# Autodesk Inventor assembly: 1001_Bias_Coil_Holder_MPSv2_v2
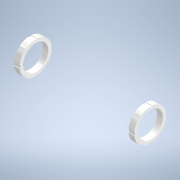
[picture p0: Inventor's stored thumbnail of the model, 180x180]
Saved by Autodesk Inventor 2021 (Build 250183000, 183)
## iProperties
Created: 2020-11-17
Part Number: 1001_Bias_Coil_Holder_MPSv2_v2
Document SubType Name: Assembly
Designer: Admin
Author: Admin
## Documents named in this file (3)
- C:\Users\Barksdale\Dropbox (MIT)\MPI Group Folder\MPS\Inventor_Parts\MPSV2\1xxx Assemblies\10xx_Coil_Positioning_Assemblies\1001_Bias_Coil_Holder_MPSv2_v2.iam
- C:\Users\Barksdale\Dropbox (MIT)\MPI Group Folder\MPS\Inventor_Parts\MPSV2\1xxx Assemblies\10xx_Coil_Positioning_Assemblies\1000_Bias_Coil_Spacers_MPSv2_v1.iam
- C:\Users\Barksdale\Dropbox (MIT)\MPI Group Folder\MPS\Inventor_Parts\MPSV2\4xxx Bias Coil\4001_Bias_Coil_Holder_Tube_Mount_Base_MPSv2_v2.ipt
## Components (10 placed, 2 different names)
1. 4001_Bias_Coil_Holder_Tube_Mount_Base_MPSv2_v2:1 — Mate:2, Mate:27, Mate:28
2. 4001_Bias_Coil_Holder_Tube_Mount_Base_MPSv2_v2:2 — Mate:2, Mate:3, Mate:4, Mate:5, Mate:6, Mate:7, Mate:8, Mate:9, Mate:10, Mate:11, Mate:12, Mate:13, Mate:14, Mate:15, Mate:16, Mate:17, Mate:18, Mate:19, Mate:20, Mate:21, Mate:22, Mate:23, Mate:24, Mate:25, Mate:26
3. 1000_Bias_Coil_Spacers_MPSv2_v1:1 [sub-assembly] — Mate:9, Mate:18, Mate:22
4. 1000_Bias_Coil_Spacers_MPSv2_v1:2 [sub-assembly] — Mate:8, Mate:12, Mate:20, Mate:27
5. 1000_Bias_Coil_Spacers_MPSv2_v1:3 [sub-assembly] — Mate:10, Mate:11, Mate:21, Mate:28
6. 1000_Bias_Coil_Spacers_MPSv2_v1:4 [sub-assembly] — Mate:7, Mate:13, Mate:19
7. 1000_Bias_Coil_Spacers_MPSv2_v1:5 [sub-assembly] — Mate:6, Mate:14, Mate:26
8. 1000_Bias_Coil_Spacers_MPSv2_v1:6 [sub-assembly] — Mate:5, Mate:15, Mate:25
9. 1000_Bias_Coil_Spacers_MPSv2_v1:7 [sub-assembly] — Mate:4, Mate:17, Mate:23
10. 1000_Bias_Coil_Spacers_MPSv2_v1:8 [sub-assembly] — Mate:3, Mate:16, Mate:24
## Relationships (27: Mate 27)
- Mate:2 (180 mm): 4001_Bias_Coil_Holder_Tube_Mount_Base_MPSv2_v2:1 ↔ 4001_Bias_Coil_Holder_Tube_Mount_Base_MPSv2_v2:2
- Mate:3: 4001_Bias_Coil_Holder_Tube_Mount_Base_MPSv2_v2:2 ↔ 1000_Bias_Coil_Spacers_MPSv2_v1:8
- Mate:4: 4001_Bias_Coil_Holder_Tube_Mount_Base_MPSv2_v2:2 ↔ 1000_Bias_Coil_Spacers_MPSv2_v1:7
- Mate:5: 4001_Bias_Coil_Holder_Tube_Mount_Base_MPSv2_v2:2 ↔ 1000_Bias_Coil_Spacers_MPSv2_v1:6
- Mate:6: 4001_Bias_Coil_Holder_Tube_Mount_Base_MPSv2_v2:2 ↔ 1000_Bias_Coil_Spacers_MPSv2_v1:5
- Mate:7: 4001_Bias_Coil_Holder_Tube_Mount_Base_MPSv2_v2:2 ↔ 1000_Bias_Coil_Spacers_MPSv2_v1:4
- Mate:8: 4001_Bias_Coil_Holder_Tube_Mount_Base_MPSv2_v2:2 ↔ 1000_Bias_Coil_Spacers_MPSv2_v1:2
- Mate:9: 4001_Bias_Coil_Holder_Tube_Mount_Base_MPSv2_v2:2 ↔ 1000_Bias_Coil_Spacers_MPSv2_v1:1
- Mate:10: 4001_Bias_Coil_Holder_Tube_Mount_Base_MPSv2_v2:2 ↔ 1000_Bias_Coil_Spacers_MPSv2_v1:3
- Mate:11: 4001_Bias_Coil_Holder_Tube_Mount_Base_MPSv2_v2:2 ↔ 1000_Bias_Coil_Spacers_MPSv2_v1:3
- Mate:12: 4001_Bias_Coil_Holder_Tube_Mount_Base_MPSv2_v2:2 ↔ 1000_Bias_Coil_Spacers_MPSv2_v1:2
- Mate:13: 4001_Bias_Coil_Holder_Tube_Mount_Base_MPSv2_v2:2 ↔ 1000_Bias_Coil_Spacers_MPSv2_v1:4
- Mate:14: 4001_Bias_Coil_Holder_Tube_Mount_Base_MPSv2_v2:2 ↔ 1000_Bias_Coil_Spacers_MPSv2_v1:5
- Mate:15: 4001_Bias_Coil_Holder_Tube_Mount_Base_MPSv2_v2:2 ↔ 1000_Bias_Coil_Spacers_MPSv2_v1:6
- Mate:16: 4001_Bias_Coil_Holder_Tube_Mount_Base_MPSv2_v2:2 ↔ 1000_Bias_Coil_Spacers_MPSv2_v1:8
- Mate:17: 4001_Bias_Coil_Holder_Tube_Mount_Base_MPSv2_v2:2 ↔ 1000_Bias_Coil_Spacers_MPSv2_v1:7
- Mate:18: 4001_Bias_Coil_Holder_Tube_Mount_Base_MPSv2_v2:2 ↔ 1000_Bias_Coil_Spacers_MPSv2_v1:1
- Mate:19: 4001_Bias_Coil_Holder_Tube_Mount_Base_MPSv2_v2:2 ↔ 1000_Bias_Coil_Spacers_MPSv2_v1:4
- Mate:20: 4001_Bias_Coil_Holder_Tube_Mount_Base_MPSv2_v2:2 ↔ 1000_Bias_Coil_Spacers_MPSv2_v1:2
- Mate:21: 4001_Bias_Coil_Holder_Tube_Mount_Base_MPSv2_v2:2 ↔ 1000_Bias_Coil_Spacers_MPSv2_v1:3
- Mate:22: 4001_Bias_Coil_Holder_Tube_Mount_Base_MPSv2_v2:2 ↔ 1000_Bias_Coil_Spacers_MPSv2_v1:1
- Mate:23: 4001_Bias_Coil_Holder_Tube_Mount_Base_MPSv2_v2:2 ↔ 1000_Bias_Coil_Spacers_MPSv2_v1:7
- Mate:24: 4001_Bias_Coil_Holder_Tube_Mount_Base_MPSv2_v2:2 ↔ 1000_Bias_Coil_Spacers_MPSv2_v1:8
- Mate:25: 4001_Bias_Coil_Holder_Tube_Mount_Base_MPSv2_v2:2 ↔ 1000_Bias_Coil_Spacers_MPSv2_v1:6
- Mate:26: 4001_Bias_Coil_Holder_Tube_Mount_Base_MPSv2_v2:2 ↔ 1000_Bias_Coil_Spacers_MPSv2_v1:5
- Mate:27: 4001_Bias_Coil_Holder_Tube_Mount_Base_MPSv2_v2:1 ↔ 1000_Bias_Coil_Spacers_MPSv2_v1:2
- Mate:28: 4001_Bias_Coil_Holder_Tube_Mount_Base_MPSv2_v2:1 ↔ 1000_Bias_Coil_Spacers_MPSv2_v1:3
